# Autodesk Inventor assembly: stemPrint
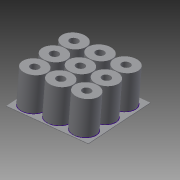
[picture p0: Inventor's stored thumbnail of the model, 180x180]
Saved by Autodesk Inventor 2014 (Build 180170000, 170)
## iProperties
Created: 2014-04-02
Part Number: stemPrint
Document SubType Name: Assembly
Designer: jferner
Author: jferner
## Documents named in this file (3)
- C:\Users\jferner\Downloads\flower\stemPrint.iam
- C:\Users\jferner\Downloads\flower\stem.ipt
- C:\Users\jferner\Downloads\flower\stemBed.ipt
## Components (10 placed, 2 different names)
1. stemBed:1 — Mate:1
2. stem:1
3. stem:2
4. stem:3
5. stem:4
6. stem:5
7. stem:6
8. stem:7 — Mate:1
9. stem:8
10. stem:9
## Component patterns: (9 elements, first: stem:1)
## Relationships (1: Mate 1)
- Mate:1: stemBed:1 ↔ stem:7
